# Autodesk Inventor assembly: 000-RZvector-arm-rotate-v1
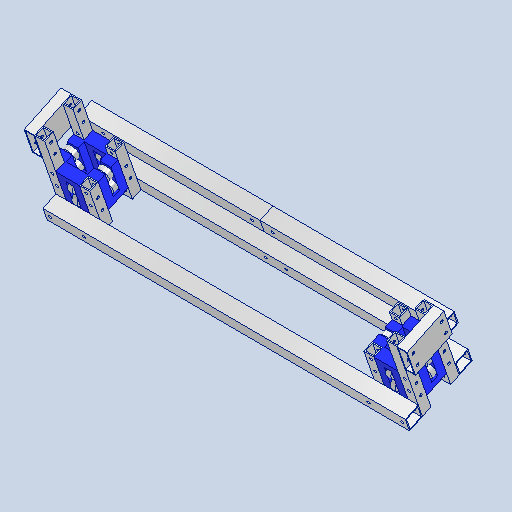
[picture p0: Inventor's stored thumbnail of the model, 512x512]
Saved by Autodesk Inventor 2025.1 (Build 291241000, 241)
## iProperties
Created: 2024-03-10
Part Number: 000-RZvector-arm-rotate-v1
Document SubType Name: Assembly
Designer: haruy
Mass: 934.228 g
Surface Area: 5002.42 cm^2
Volume: 469.897 cm^3
Density: 1.98815 g/cm^3
Author: haruy
## Documents named in this file (4)
- C:\Users\haruy\Documents\ロボコン\NHK2025\cad\nagahisa\dribl\R2-Rzvector\000-RZvector-arm-rotate-v1.iam
- C:\Users\haruy\Documents\ロボコン\NHK2025\cad\nagahisa\dribl\R2-Rzvector\RZvector-arm-rotate-v1-ASP-Base.ipt
- C:\Users\haruy\Documents\ロボコン\NHK2025\cad\nagahisa\dribl\R2-Rzvector\RZvector-Srunit-v2-ASP-Base.ipt
- C:\Users\haruy\Documents\ロボコン\NHK2025\cad\nagahisa\dribl\R2-Rzvector\RZvector-Srunit-v2-3DP-Spacer.ipt
## Components (4 placed, 3 different names)
1. RZvector-arm-rotate-v1-ASP-Base:1 — 挿入:35, 挿入:36
2. RZvector-Srunit-v2-ASP-Base:1 — 挿入:35, 挿入:36, 挿入:37, 挿入:38, 挿入:39, 挿入:40
3. RZvector-Srunit-v2-3DP-Spacer:1 — 挿入:37, 挿入:38
4. RZvector-Srunit-v2-3DP-Spacer:2 — 挿入:39, 挿入:40
## Relationships (6: Insert 6)
- 挿入:35 [Insert]: RZvector-arm-rotate-v1-ASP-Base:1 ↔ RZvector-Srunit-v2-ASP-Base:1
- 挿入:36 [Insert]: RZvector-arm-rotate-v1-ASP-Base:1 ↔ RZvector-Srunit-v2-ASP-Base:1
- 挿入:37 [Insert]: RZvector-Srunit-v2-ASP-Base:1 ↔ RZvector-Srunit-v2-3DP-Spacer:1
- 挿入:38 [Insert]: RZvector-Srunit-v2-ASP-Base:1 ↔ RZvector-Srunit-v2-3DP-Spacer:1
- 挿入:39 [Insert]: RZvector-Srunit-v2-ASP-Base:1 ↔ RZvector-Srunit-v2-3DP-Spacer:2
- 挿入:40 [Insert]: RZvector-Srunit-v2-ASP-Base:1 ↔ RZvector-Srunit-v2-3DP-Spacer:2
